# Autodesk Inventor assembly: 組合檔
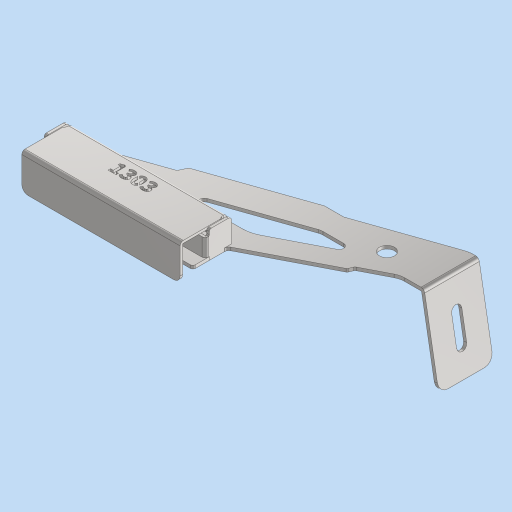
[picture p0: Inventor's stored thumbnail of the model, 512x512]
Saved by Autodesk Inventor 2023 (Build 270158000, 158)
## iProperties
Created: 2015-11-28
Part Number: 組合檔
Document SubType Name: Assembly
Designer: 設計製圖
Author: 設計製圖
## Documents named in this file (3)
- D:\資料庫\設計-工業3D\【May club 】\得利卡-車頂燈架\模型、圖面\成品版本\短-車頂燈架-組合(v220714)\吊架-短(R)-完整(v220714).iam
- D:\資料庫\設計-工業3D\【May club 】\得利卡-車頂燈架\模型、圖面\成品版本\短-車頂燈架-組合(v220714)\吊架-短(R) - 焊接組合(v220714).iam
- D:\資料庫\設計-工業3D\【May club 】\得利卡-車頂燈架\模型、圖面\成品版本\短-車頂燈架-組合(v220714)\ㄇ槽- 焊接組合(v220714).iam
## Components (2 placed, 2 different names)
1. 吊架-短(R) - 焊接組合(v220714):1 [sub-assembly] — 貼合:1, 貼合:2
2. ㄇ槽- 焊接組合(v220714):1 [sub-assembly] — 貼合:1, 貼合:2
## Relationships (3: Mate 2, Flush 1)
- 貼合:1 [Mate]: 吊架-短(R) - 焊接組合(v220714):1 ↔ ㄇ槽- 焊接組合(v220714):1
- 貼合:2 [Mate]: 吊架-短(R) - 焊接組合(v220714):1 ↔ ㄇ槽- 焊接組合(v220714):1
- 齊平:1 [Flush] (-120 mm)
